# Autodesk Inventor assembly: 20mm Gantry Set
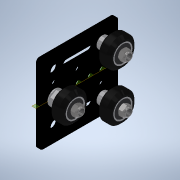
[picture p0: Inventor's stored thumbnail of the model, 180x180]
Saved by Autodesk Inventor 2020.3 (Build 243373000, 373)
## iProperties
Created: 2016-04-10
Part Number: 20mm Gantry Set
Document SubType Name: Assembly
Designer: Ben
Mass: 48.8675 g
Surface Area: 277.219 cm^2
Volume: 30.9657 cm^3
Density: 1.57812 g/cm^3
Author: Ben
## Documents named in this file (5)
- C:\Users\juanp\Desktop\Diseño EVA\Actuador Lineal\Placas deslizantes\20mm Gantry Set.iam
- C:\Users\juanp\Desktop\Diseño EVA\Actuador Lineal\Placas deslizantes\V-Slot Gantry Plate 20mm.ipt
- C:\Users\juanp\Desktop\Diseño EVA\Actuador Lineal\Placas deslizantes\V-Wheel Solid Wheel.iam
- C:\Users\juanp\Desktop\Diseño EVA\Actuador Lineal\Placas deslizantes\V-Wheel Solid Wheel - spacer.iam
- C:\Users\juanp\Desktop\Diseño EVA\Actuador Lineal\Placas deslizantes\M5 Nylock.ipt
## Components (7 placed, 4 different names)
1. V-Slot Gantry Plate 20mm:1 — Mate:34, Mate:35, Mate:36, Mate:41, Angle:2, Mate:54, Mate:55, Mate:56, Mate:57, Mate:58, Mate:68
2. V-Wheel Solid Wheel - spacer:2 [sub-assembly] — Mate:24, Mate:41, Mate:55
3. M5 Nylock:4 — Mate:24, Angle:2, Mate:56
4. V-Wheel Solid Wheel - spacer:3 [sub-assembly] — Mate:54, Mate:57
5. M5 Nylock:5 — Mate:58
6. V-Wheel Solid Wheel:5 [sub-assembly] — Mate:68
7. M5 Nylock:6
## Relationships (15: Mate 13, Flush 1, Angle 1)
- Mate:24: V-Wheel Solid Wheel - spacer:2 ↔ M5 Nylock:4
- Flush:2
- Mate:34: V-Slot Gantry Plate 20mm:1
- Mate:35: V-Slot Gantry Plate 20mm:1
- Mate:36: V-Slot Gantry Plate 20mm:1
- Mate:41: V-Slot Gantry Plate 20mm:1 ↔ V-Wheel Solid Wheel - spacer:2
- Angle:2 (0 deg): V-Slot Gantry Plate 20mm:1 ↔ M5 Nylock:4
- [Mate]: V-Wheel Solid Wheel - spacer:3 ↔ M5 Nylock:5
- Mate:54: V-Slot Gantry Plate 20mm:1 ↔ V-Wheel Solid Wheel - spacer:3
- Mate:55: V-Slot Gantry Plate 20mm:1 ↔ V-Wheel Solid Wheel - spacer:2
- Mate:56: V-Slot Gantry Plate 20mm:1 ↔ M5 Nylock:4
- Mate:57: V-Slot Gantry Plate 20mm:1 ↔ V-Wheel Solid Wheel - spacer:3
- Mate:58: V-Slot Gantry Plate 20mm:1 ↔ M5 Nylock:5
- [Mate]: V-Wheel Solid Wheel:5 ↔ M5 Nylock:6
- Mate:68: V-Slot Gantry Plate 20mm:1 ↔ V-Wheel Solid Wheel:5
## Named parameters: d60_d23 = 0 mm, d75_d22 = 0 mm
